# Autodesk Inventor assembly: ruka_backup
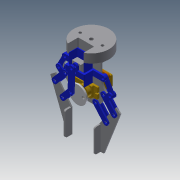
[picture p0: Inventor's stored thumbnail of the model, 180x180]
Saved by Autodesk Inventor 2013 (Build 170138000, 138)
## iProperties
Created: 2013-02-02
Part Number: ruka_backup
Document SubType Name: Assembly
Designer: idle-rug
Author: idle-rug
## Documents named in this file (16)
- C:\Users\Petr\Documents\Inventor\robotic arm\ruka_backup.iam
- C:\Users\Petr\Documents\Inventor\robotic arm\ruka_zak, deska.ipt
- C:\Users\Petr\Documents\Inventor\robotic arm\ruka_tahlo.ipt
- C:\Users\Petr\Documents\Inventor\robotic arm\tahlo3.ipt
- C:\Users\Petr\Documents\Inventor\robotic arm\kolejnicka_ruka.ipt
- C:\Users\Petr\Documents\Inventor\robotic arm\kolejnicka_ruka_druha_cast.ipt
- C:\Users\Petr\Documents\Inventor\robotic arm\tahlo6.ipt
- C:\Users\Petr\Documents\Inventor\robotic arm\tahlo5(b).ipt
- C:\Users\Petr\Documents\Inventor\robotic arm\micro_servo.ipt
- C:\Users\Petr\Documents\Inventor\robotic arm\paka2_micro.ipt
- C:\Users\Petr\Documents\Inventor\robotic arm\tahlo5.ipt
- C:\Users\Petr\Documents\Inventor\robotic arm\tahlo7.ipt
- C:\Users\Petr\Documents\Inventor\robotic arm\packa_prava.ipt
- C:\Users\Petr\Documents\Inventor\robotic arm\pracka_leva1.ipt
- C:\Users\Petr\Documents\Inventor\robotic arm\ruka_lozisko.ipt
- C:\Users\Petr\Documents\Inventor\robotic arm\rameno\paka_packa.ipt
## Components (22 placed, 15 different names)
1. ruka_zak, deska:1 — Mate:141, Mate:142, Mate:169, Mate:196, Mate:199, Mate:230, Mate:231, Mate:235, Mate:238, Mate:250, Mate:277, Mate:278, Mate:279, Mate:280, Mate:297, Mate:298, Mate:299, Mate:322, Mate:323, Mate:324, Mate:325, Mate:326, Mate:327, Mate:328, Mate:330, Mate:344, Mate:345, Mate:346, Mate:347, Mate:348, Mate:349, Mate:350
2. ruka_tahlo:1 — Mate:142, Mate:169, Mate:313
3. ruka_tahlo:2 — Mate:141, Mate:230, Mate:231, Mate:314
4. ruka_tahlo:3 — Mate:199, Mate:310, Mate:318, Mate:328
5. ruka_tahlo:4 — Mate:196, Mate:311, Mate:317, Mate:330
6. tahlo3:2 — Mate:235, Mate:319, Mate:327, Mate:329, Mate:335
7. tahlo3:3 — Mate:238, Mate:316, Mate:320, Mate:322, Mate:342
8. kolejnicka_ruka:1 — Mate:243, Mate:244, Mate:297, Mate:298, Mate:323
9. kolejnicka_ruka_druha_cast:1 — Mate:243, Mate:244, Mate:304, Mate:305, Mate:306
10. micro_servo:1 — Mate:250, Mate:251, Mate:252, Mate:324, Mate:325, Mate:326
11. paka2_micro:1 — Mate:251, Mate:252, Mate:273, Mate:274
12. tahlo5:1 — Mate:273, Mate:274, Mate:309
13. tahlo3:4 — Mate:277, Mate:280, Mate:312, Mate:336
14. tahlo3:5 — Mate:278, Mate:279, Mate:315, Mate:341
15. tahlo7:1 — Mate:299, Mate:332, Mate:334, Mate:337, Mate:339
16. tahlo6:1 — Mate:304, Mate:305, Mate:306, Mate:309, Mate:332, Mate:334, Mate:338, Mate:340
17. packa_prava:1 — Mate:310, Mate:312, Mate:313, Mate:318, Mate:319, Mate:329
18. pracka_leva1:1 — Mate:311, Mate:314, Mate:315, Mate:316, Mate:317
19. tahlo5(b):4 — Mate:320, Mate:339, Mate:340, Mate:341, Mate:342
20. tahlo5(b):5 — Mate:335, Mate:336, Mate:337, Mate:338
21. ruka_lozisko:1 — Mate:344, Mate:345, Mate:346, Mate:347
22. paka_packa:1 — Mate:348, Mate:349, Mate:350
## Relationships (64: Mate 64)
- Mate:141: ruka_zak, deska:1 ↔ ruka_tahlo:2
- Mate:142: ruka_zak, deska:1 ↔ ruka_tahlo:1
- Mate:169: ruka_zak, deska:1 ↔ ruka_tahlo:1
- Mate:196: ruka_zak, deska:1 ↔ ruka_tahlo:4
- Mate:199: ruka_zak, deska:1 ↔ ruka_tahlo:3
- Mate:230: ruka_zak, deska:1 ↔ ruka_tahlo:2
- Mate:231: ruka_zak, deska:1 ↔ ruka_tahlo:2
- Mate:235: ruka_zak, deska:1 ↔ tahlo3:2
- Mate:238: ruka_zak, deska:1 ↔ tahlo3:3
- Mate:243 (3 mm): kolejnicka_ruka:1 ↔ kolejnicka_ruka_druha_cast:1
- Mate:244: kolejnicka_ruka:1 ↔ kolejnicka_ruka_druha_cast:1
- Mate:250: ruka_zak, deska:1 ↔ micro_servo:1
- Mate:251: micro_servo:1 ↔ paka2_micro:1
- Mate:252: micro_servo:1 ↔ paka2_micro:1
- Mate:273: paka2_micro:1 ↔ tahlo5:1
- Mate:274: paka2_micro:1 ↔ tahlo5:1
- Mate:277: ruka_zak, deska:1 ↔ tahlo3:4
- Mate:278: ruka_zak, deska:1 ↔ tahlo3:5
- Mate:279: ruka_zak, deska:1 ↔ tahlo3:5
- Mate:280: ruka_zak, deska:1 ↔ tahlo3:4
- Mate:297: ruka_zak, deska:1 ↔ kolejnicka_ruka:1
- Mate:298: ruka_zak, deska:1 ↔ kolejnicka_ruka:1
- Mate:299: ruka_zak, deska:1 ↔ tahlo7:1
- Mate:304: kolejnicka_ruka_druha_cast:1 ↔ tahlo6:1
- Mate:305: kolejnicka_ruka_druha_cast:1 ↔ tahlo6:1
- Mate:306: kolejnicka_ruka_druha_cast:1 ↔ tahlo6:1
- Mate:309: tahlo5:1 ↔ tahlo6:1
- Mate:310: ruka_tahlo:3 ↔ packa_prava:1
- Mate:311: ruka_tahlo:4 ↔ pracka_leva1:1
- Mate:312: tahlo3:4 ↔ packa_prava:1
- Mate:313: ruka_tahlo:1 ↔ packa_prava:1
- Mate:314: ruka_tahlo:2 ↔ pracka_leva1:1
- Mate:315: tahlo3:5 ↔ pracka_leva1:1
- Mate:316: tahlo3:3 ↔ pracka_leva1:1
- Mate:317: ruka_tahlo:4 ↔ pracka_leva1:1
- Mate:318: ruka_tahlo:3 ↔ packa_prava:1
- Mate:319: tahlo3:2 ↔ packa_prava:1
- Mate:320: tahlo3:3 ↔ tahlo5(b):4
- Mate:322: ruka_zak, deska:1 ↔ tahlo3:3
- Mate:323: ruka_zak, deska:1 ↔ kolejnicka_ruka:1
- Mate:324: ruka_zak, deska:1 ↔ micro_servo:1
- Mate:325: ruka_zak, deska:1 ↔ micro_servo:1
- Mate:326: ruka_zak, deska:1 ↔ micro_servo:1
- Mate:327: ruka_zak, deska:1 ↔ tahlo3:2
- Mate:328: ruka_zak, deska:1 ↔ ruka_tahlo:3
- Mate:329: tahlo3:2 ↔ packa_prava:1
- Mate:330: ruka_zak, deska:1 ↔ ruka_tahlo:4
- Mate:332: tahlo7:1 ↔ tahlo6:1
- Mate:334: tahlo7:1 ↔ tahlo6:1
- Mate:335: tahlo3:2 ↔ tahlo5(b):5
- Mate:336: tahlo3:4 ↔ tahlo5(b):5
- Mate:337: tahlo7:1 ↔ tahlo5(b):5
- Mate:338: tahlo6:1 ↔ tahlo5(b):5
- Mate:339: tahlo7:1 ↔ tahlo5(b):4
- Mate:340: tahlo6:1 ↔ tahlo5(b):4
- Mate:341: tahlo3:5 ↔ tahlo5(b):4
- Mate:342: tahlo3:3 ↔ tahlo5(b):4
- Mate:344: ruka_zak, deska:1 ↔ ruka_lozisko:1
- Mate:345: ruka_zak, deska:1 ↔ ruka_lozisko:1
- Mate:346: ruka_zak, deska:1 ↔ ruka_lozisko:1
- Mate:347: ruka_zak, deska:1 ↔ ruka_lozisko:1
- Mate:348: ruka_zak, deska:1 ↔ paka_packa:1
- Mate:349: ruka_zak, deska:1 ↔ paka_packa:1
- Mate:350: ruka_zak, deska:1 ↔ paka_packa:1
